# Autodesk Inventor assembly: 42146-10
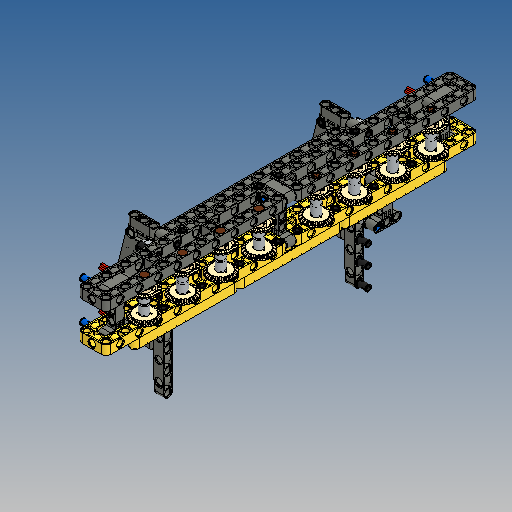
[picture p0: Inventor's stored thumbnail of the model, 512x512]
Saved by Autodesk Inventor 2025 (Build 290162010, 162A)
## iProperties
Created: 2024-11-16
Part Number: 42146-10
Material: Generisch
Document SubType Name: Assembly
Designer: hp.muther
Author: hp.muther
## Documents named in this file (16)
- D:\Inventor\Projekte\Muther\LEGO Technic\LEGO Technik - Raupenkran LR 13000 (42146)\42146-01-10.iam
- D:\Inventor\Projekte\Muther\LEGO Technic\LEGO Pieces\Rahmen, T-Stücke\67491-Yellow.ipt
- D:\Inventor\Projekte\Muther\LEGO Technic\LEGO Pieces\Pin's\6558-Blue.ipt
- D:\Inventor\Projekte\Muther\LEGO Technic\LEGO Pieces\Pin's\11214-Red.ipt
- D:\Inventor\Projekte\Muther\LEGO Technic\LEGO Pieces\Achsen\15462-ReddishBrown.ipt
- D:\Inventor\Projekte\Muther\LEGO Technic\LEGO Pieces\Zahnrad\32198-Tan.ipt
- D:\Inventor\Projekte\Muther\LEGO Technic\LEGO Pieces\Rund\62462-LtBluishGray.ipt
- D:\Inventor\Projekte\Muther\LEGO Technic\LEGO Pieces\Rahmen, T-Stücke\67491-DkBluishGray.ipt
- D:\Inventor\Projekte\Muther\LEGO Technic\LEGO Pieces\Rahmen, T-Stücke\14720-DkBluishGray.ipt
- D:\Inventor\Projekte\Muther\LEGO Technic\LEGO Pieces\Lochbalken\32525-Yellow.ipt
- D:\Inventor\Projekte\Muther\LEGO Technic\LEGO Pieces\Pin's\2780-Black.ipt
- D:\Inventor\Projekte\Muther\LEGO Technic\LEGO Pieces\Pin's\32054-LtBluishGray.ipt
- D:\Inventor\Projekte\Muther\LEGO Technic\LEGO Pieces\Paneelen\18945-DkBluishGray.ipt
- D:\Inventor\Projekte\Muther\LEGO Technic\LEGO Pieces\Pin's\43093-Blue.ipt
- D:\Inventor\Projekte\Muther\LEGO Technic\LEGO Pieces\Lochbalken\43857-LtBluishGray.ipt
- D:\Inventor\Projekte\Muther\LEGO Technic\LEGO Pieces\Lochbalken\771710-DkBluishGray.ipt
## Components (94 placed, 15 different names)
1. 67491-Yellow:1 — Einfügen:1, Einfügen:2, Einfügen:7, Einfügen:8, Einfügen:9, Einfügen:10, Passend:1, Einfügen:23, Einfügen:53, Einfügen:55, Passend:17, Einfügen:56, Passend:18, Einfügen:57, Einfügen:58
2. 6558-Blue:1 — Einfügen:2, Passend:3
3. 11214-Red:1 — Einfügen:1, Passend:2
4. 15462-ReddishBrown:1 — Einfügen:3
5. 32198-Tan:1 — Einfügen:3, Einfügen:10, Einfügen:18
6. 15462-ReddishBrown:2
7. 32198-Tan:2 — Einfügen:9, Einfügen:17
8. 15462-ReddishBrown:3
9. 32198-Tan:3 — Einfügen:8, Einfügen:16
10. 15462-ReddishBrown:4
11. 32198-Tan:4 — Einfügen:7, Einfügen:15
12. 32198-Tan:5 — Einfügen:11
13. 62462-LtBluishGray:1 — Einfügen:11, Einfügen:18
14. 32198-Tan:6
15. 62462-LtBluishGray:2 — Einfügen:17
16. 32198-Tan:7
17. 62462-LtBluishGray:3 — Einfügen:16
18. 32198-Tan:8
19. 62462-LtBluishGray:4 — Einfügen:15
20. 14720-DkBluishGray:1 — Passend:1, Passend:2, Passend:3, Passend:4, Passend:5, Passend:6
21. 67491-DkBluishGray:1 — Passend:4, Passend:7, Passend:19, Einfügen:59, Einfügen:75
22. 6558-Blue:2 — Passend:5
23. 11214-Red:2 — Passend:6
24. 6558-Blue:3 — Einfügen:21, Passend:7, Passend:14
25. 14720-DkBluishGray:2 — Einfügen:21, Einfügen:22, Einfügen:44
26. 6558-Blue:4 — Einfügen:22, Einfügen:23
27. 67491-DkBluishGray:2 — Passend:14, Einfügen:64, Einfügen:82, Einfügen:89
28. 6558-Blue:5
29. 11214-Red:3
30. 15462-ReddishBrown:5
31. 32198-Tan:9
32. 15462-ReddishBrown:6
33. 32198-Tan:10
34. 15462-ReddishBrown:7
35. 32198-Tan:11
36. 15462-ReddishBrown:8
37. 32198-Tan:12
38. 32198-Tan:13
39. 62462-LtBluishGray:5
40. 32198-Tan:14
41. 62462-LtBluishGray:6
42. 32198-Tan:15
43. 62462-LtBluishGray:7
44. 32198-Tan:16
45. 62462-LtBluishGray:8
46. 14720-DkBluishGray:3
47. 67491-Yellow:3 — Einfügen:44, Passend:15, Einfügen:54, Passend:16, Passend:23, Einfügen:90
48. 6558-Blue:6
49. 11214-Red:4
50. 32525-Yellow:1 — Einfügen:49, Einfügen:50, Einfügen:55
51. 32525-Yellow:2 — Einfügen:45, Einfügen:46, Einfügen:47, Einfügen:48, Einfügen:53
52. 2780-Black:1 — Einfügen:50, Passend:17
53. 2780-Black:2 — Einfügen:49
54. 2780-Black:3 — Einfügen:47
55. 2780-Black:4 — Einfügen:46
56. 2780-Black:5 — Einfügen:48
57. 2780-Black:6 — Einfügen:45, Passend:15
58. 2780-Black:7 — Einfügen:59
59. 6558-Blue:7 — Einfügen:58
60. 11214-Red:5 — Einfügen:57
61. 2780-Black:8 — Einfügen:71, Passend:21
62. 2780-Black:9 — Einfügen:78, Passend:22
63. 2780-Black:10 — Einfügen:80
64. 2780-Black:11 — Einfügen:72
65. 2780-Black:12 — Einfügen:69, Passend:20
66. 2780-Black:13 — Einfügen:67
67. 2780-Black:14 — Einfügen:66
68. 2780-Black:15 — Einfügen:68
69. 32054-LtBluishGray:1 — Einfügen:65, Einfügen:74
70. 32525-Yellow:3 — Einfügen:52, Einfügen:54
71. 2780-Black:16 — Einfügen:52
72. 2780-Black:17 — Passend:16
73. 14720-DkBluishGray:4 — Einfügen:56, Passend:18, Einfügen:76
74. 67491-DkBluishGray:3 — Einfügen:60, Einfügen:61, Einfügen:62, Einfügen:63, Einfügen:64
75. 2780-Black:18 — Einfügen:60, Passend:19
76. 2780-Black:19 — Einfügen:63
77. 2780-Black:20 — Einfügen:62
78. 2780-Black:21 — Einfügen:61
79. 771710-DkBluishGray:1 — Einfügen:65, Einfügen:66, Einfügen:67, Einfügen:68, Einfügen:69, Einfügen:70, Einfügen:75, Einfügen:79
80. 32525-Yellow:4 — Einfügen:73, Passend:21
81. 18945-DkBluishGray:1 — Einfügen:70, Passend:20, Einfügen:71, Einfügen:72, Einfügen:73, Passend:22
82. 43093-Blue:1 — Einfügen:74, Einfügen:76
83. 6558-Blue:8 — Einfügen:77
84. 43857-LtBluishGray:1 — Einfügen:77, Einfügen:78, Einfügen:79
85. 771710-DkBluishGray:2 — Einfügen:80, Einfügen:81, Einfügen:82, Einfügen:83, Einfügen:84, Einfügen:85, Einfügen:88
86. 18945-DkBluishGray:2 — Einfügen:85, Passend:24, Passend:25
87. 2780-Black:22 — Einfügen:83
88. 2780-Black:23 — Einfügen:84, Passend:24
89. 6558-Blue:9 — Einfügen:81, Passend:23
90. 2780-Black:24 — Passend:25
91. 6558-Blue:10
92. 43857-LtBluishGray:2 — Einfügen:88
93. 2780-Black:25 — Einfügen:89
94. 2780-Black:26 — Einfügen:90
## Relationships (115: Insert 90, Mate 25)
- Einfügen:1 [Insert]: 67491-Yellow:1 ↔ 11214-Red:1
- Einfügen:2 [Insert]: 67491-Yellow:1 ↔ 6558-Blue:1
- Einfügen:3 [Insert] (7.2 mm): 15462-ReddishBrown:1 ↔ 32198-Tan:1
- [Insert] (7.2 mm): 15462-ReddishBrown:2 ↔ 32198-Tan:2
- [Insert] (7.2 mm): 15462-ReddishBrown:3 ↔ 32198-Tan:3
- [Insert] (7.2 mm): 15462-ReddishBrown:4 ↔ 32198-Tan:4
- Einfügen:7 [Insert]: 67491-Yellow:1 ↔ 32198-Tan:4
- Einfügen:8 [Insert]: 67491-Yellow:1 ↔ 32198-Tan:3
- Einfügen:9 [Insert]: 67491-Yellow:1 ↔ 32198-Tan:2
- Einfügen:10 [Insert]: 67491-Yellow:1 ↔ 32198-Tan:1
- Einfügen:11 [Insert]: 32198-Tan:5 ↔ 62462-LtBluishGray:1
- [Insert]: 32198-Tan:6 ↔ 62462-LtBluishGray:2
- [Insert]: 32198-Tan:7 ↔ 62462-LtBluishGray:3
- [Insert]: 32198-Tan:8 ↔ 62462-LtBluishGray:4
- Einfügen:15 [Insert]: 32198-Tan:4 ↔ 62462-LtBluishGray:4
- Einfügen:16 [Insert]: 32198-Tan:3 ↔ 62462-LtBluishGray:3
- Einfügen:17 [Insert]: 32198-Tan:2 ↔ 62462-LtBluishGray:2
- Einfügen:18 [Insert]: 32198-Tan:1 ↔ 62462-LtBluishGray:1
- Passend:1 [Mate]: 67491-Yellow:1 ↔ 14720-DkBluishGray:1
- Passend:2 [Mate]: 11214-Red:1 ↔ 14720-DkBluishGray:1
- Passend:3 [Mate]: 6558-Blue:1 ↔ 14720-DkBluishGray:1
- [Insert]: 67491-DkBluishGray:1 ↔ 11214-Red:2
- [Insert]: 67491-DkBluishGray:1 ↔ 6558-Blue:2
- Passend:4 [Mate]: 14720-DkBluishGray:1 ↔ 67491-DkBluishGray:1
- Passend:5 [Mate]: 14720-DkBluishGray:1 ↔ 6558-Blue:2
- Passend:6 [Mate]: 14720-DkBluishGray:1 ↔ 11214-Red:2
- Einfügen:21 [Insert]: 6558-Blue:3 ↔ 14720-DkBluishGray:2
- Einfügen:22 [Insert]: 14720-DkBluishGray:2 ↔ 6558-Blue:4
- Einfügen:23 [Insert]: 67491-Yellow:1 ↔ 6558-Blue:4
- Passend:7 [Mate]: 67491-DkBluishGray:1 ↔ 6558-Blue:3
- [Insert]: 67491-DkBluishGray:2 ↔ 11214-Red:3
- [Insert]: 67491-DkBluishGray:2 ↔ 6558-Blue:5
- [Insert] (7.2 mm): 15462-ReddishBrown:5 ↔ 32198-Tan:9
- [Insert] (7.2 mm): 15462-ReddishBrown:6 ↔ 32198-Tan:10
- [Insert] (7.2 mm): 15462-ReddishBrown:7 ↔ 32198-Tan:11
- [Insert] (7.2 mm): 15462-ReddishBrown:8 ↔ 32198-Tan:12
- [Insert]: 67491-DkBluishGray:2 ↔ 32198-Tan:12
- [Insert]: 67491-DkBluishGray:2 ↔ 32198-Tan:11
- [Insert]: 67491-DkBluishGray:2 ↔ 32198-Tan:10
- [Insert]: 67491-DkBluishGray:2 ↔ 32198-Tan:9
- [Insert]: 32198-Tan:13 ↔ 62462-LtBluishGray:5
- [Insert]: 32198-Tan:14 ↔ 62462-LtBluishGray:6
- [Insert]: 32198-Tan:15 ↔ 62462-LtBluishGray:7
- [Insert]: 32198-Tan:16 ↔ 62462-LtBluishGray:8
- [Insert]: 32198-Tan:12 ↔ 62462-LtBluishGray:8
- [Insert]: 32198-Tan:11 ↔ 62462-LtBluishGray:7
- [Insert]: 32198-Tan:10 ↔ 62462-LtBluishGray:6
- [Insert]: 32198-Tan:9 ↔ 62462-LtBluishGray:5
- [Mate]: 67491-DkBluishGray:2 ↔ 14720-DkBluishGray:3
- [Mate]: 11214-Red:3 ↔ 14720-DkBluishGray:3
- [Mate]: 6558-Blue:5 ↔ 14720-DkBluishGray:3
- [Insert]: 67491-Yellow:3 ↔ 11214-Red:4
- [Insert]: 67491-Yellow:3 ↔ 6558-Blue:6
- [Mate]: 14720-DkBluishGray:3 ↔ 67491-Yellow:3
- [Mate]: 14720-DkBluishGray:3 ↔ 6558-Blue:6
- [Mate]: 14720-DkBluishGray:3 ↔ 11214-Red:4
- Einfügen:44 [Insert]: 14720-DkBluishGray:2 ↔ 67491-Yellow:3
- Passend:14 [Mate]: 6558-Blue:3 ↔ 67491-DkBluishGray:2
- Einfügen:45 [Insert]: 32525-Yellow:2 ↔ 2780-Black:6
- Einfügen:46 [Insert]: 32525-Yellow:2 ↔ 2780-Black:4
- Einfügen:47 [Insert]: 32525-Yellow:2 ↔ 2780-Black:3
- Einfügen:48 [Insert]: 32525-Yellow:2 ↔ 2780-Black:5
- Einfügen:49 [Insert]: 32525-Yellow:1 ↔ 2780-Black:2
- Einfügen:50 [Insert]: 32525-Yellow:1 ↔ 2780-Black:1
- [Insert]: 32525-Yellow:3 ↔ 2780-Black:17
- Einfügen:52 [Insert]: 32525-Yellow:3 ↔ 2780-Black:16
- Einfügen:53 [Insert]: 67491-Yellow:1 ↔ 32525-Yellow:2
- Passend:15 [Mate]: 67491-Yellow:3 ↔ 2780-Black:6
- Einfügen:54 [Insert]: 67491-Yellow:3 ↔ 32525-Yellow:3
- Passend:16 [Mate]: 67491-Yellow:3 ↔ 2780-Black:17
- Einfügen:55 [Insert]: 67491-Yellow:1 ↔ 32525-Yellow:1
- Passend:17 [Mate]: 67491-Yellow:1 ↔ 2780-Black:1
- Einfügen:56 [Insert]: 67491-Yellow:1 ↔ 14720-DkBluishGray:4
- Passend:18 [Mate]: 67491-Yellow:1 ↔ 14720-DkBluishGray:4
- Einfügen:57 [Insert]: 67491-Yellow:1 ↔ 11214-Red:5
- Einfügen:58 [Insert]: 67491-Yellow:1 ↔ 6558-Blue:7
- Einfügen:59 [Insert]: 67491-DkBluishGray:1 ↔ 2780-Black:7
- Einfügen:60 [Insert]: 67491-DkBluishGray:3 ↔ 2780-Black:18
- Einfügen:61 [Insert]: 67491-DkBluishGray:3 ↔ 2780-Black:21
- Einfügen:62 [Insert]: 67491-DkBluishGray:3 ↔ 2780-Black:20
- Einfügen:63 [Insert]: 67491-DkBluishGray:3 ↔ 2780-Black:19
- Einfügen:64 [Insert]: 67491-DkBluishGray:2 ↔ 67491-DkBluishGray:3
- Passend:19 [Mate]: 67491-DkBluishGray:1 ↔ 2780-Black:18
- Einfügen:65 [Insert]: 32054-LtBluishGray:1 ↔ 771710-DkBluishGray:1
- Einfügen:66 [Insert]: 2780-Black:14 ↔ 771710-DkBluishGray:1
- Einfügen:67 [Insert]: 2780-Black:13 ↔ 771710-DkBluishGray:1
- Einfügen:68 [Insert]: 2780-Black:15 ↔ 771710-DkBluishGray:1
- Einfügen:69 [Insert]: 2780-Black:12 ↔ 771710-DkBluishGray:1
- Einfügen:70 [Insert]: 771710-DkBluishGray:1 ↔ 18945-DkBluishGray:1
- Passend:20 [Mate]: 2780-Black:12 ↔ 18945-DkBluishGray:1
- Einfügen:71 [Insert]: 2780-Black:8 ↔ 18945-DkBluishGray:1
- Einfügen:72 [Insert]: 2780-Black:11 ↔ 18945-DkBluishGray:1
- Einfügen:73 [Insert]: 32525-Yellow:4 ↔ 18945-DkBluishGray:1
- Passend:21 [Mate]: 2780-Black:8 ↔ 32525-Yellow:4
- Einfügen:74 [Insert]: 32054-LtBluishGray:1 ↔ 43093-Blue:1
- Einfügen:75 [Insert]: 67491-DkBluishGray:1 ↔ 771710-DkBluishGray:1
- Einfügen:76 [Insert]: 14720-DkBluishGray:4 ↔ 43093-Blue:1
- Einfügen:77 [Insert]: 6558-Blue:8 ↔ 43857-LtBluishGray:1
- Einfügen:78 [Insert]: 2780-Black:9 ↔ 43857-LtBluishGray:1
- Einfügen:79 [Insert]: 771710-DkBluishGray:1 ↔ 43857-LtBluishGray:1
- Passend:22 [Mate]: 2780-Black:9 ↔ 18945-DkBluishGray:1
- Einfügen:80 [Insert]: 2780-Black:10 ↔ 771710-DkBluishGray:2
- Einfügen:81 [Insert]: 771710-DkBluishGray:2 ↔ 6558-Blue:9
- Einfügen:82 [Insert]: 67491-DkBluishGray:2 ↔ 771710-DkBluishGray:2
- Passend:23 [Mate]: 67491-Yellow:3 ↔ 6558-Blue:9
- Einfügen:83 [Insert]: 771710-DkBluishGray:2 ↔ 2780-Black:22
- Einfügen:84 [Insert]: 771710-DkBluishGray:2 ↔ 2780-Black:23
- Einfügen:85 [Insert]: 771710-DkBluishGray:2 ↔ 18945-DkBluishGray:2
- Passend:24 [Mate]: 18945-DkBluishGray:2 ↔ 2780-Black:23
- [Insert]: 6558-Blue:10 ↔ 43857-LtBluishGray:2
- [Insert]: 2780-Black:24 ↔ 43857-LtBluishGray:2
- Einfügen:88 [Insert]: 771710-DkBluishGray:2 ↔ 43857-LtBluishGray:2
- Passend:25 [Mate]: 18945-DkBluishGray:2 ↔ 2780-Black:24
- Einfügen:89 [Insert]: 67491-DkBluishGray:2 ↔ 2780-Black:25
- Einfügen:90 [Insert]: 67491-Yellow:3 ↔ 2780-Black:26
## Named parameters: d3_d2 = 7.2 mm, d4_d2 = 7.2 mm, d5_d2 = 7.2 mm, d11_d10 = 0 mm, d12_d10 = 0 mm, d13_d10 = 0 mm, d21_d0 = 0 mm, d22_d1 = 0 mm, d26_d20 = 0 mm, d27_d24 = 0 mm, d30_d2 = 7.2 mm, d31_d3_d2 = 7.2 mm, d32_d4_d2 = 7.2 mm, d33_d5_d2 = 7.2 mm, d34_d6 = 0 mm, d35_d7 = 0 mm, d36_d8 = 0 mm, d37_d9 = 0 mm, d38_d10 = 0 mm, d39_d11_d10 = 0 mm, d40_d12_d10 = 0 mm, d41_d13_d10 = 0 mm, d42_d14 = 0 mm, d43_d15 = 0 mm, d44_d16 = 0 mm, d45_d17 = 0 mm, d46_d18 = 0 mm, d47_d19 = 0 mm, d48_d20 = 0 mm, d49_d21_d0 = 0 mm, d50_d22_d1 = 0 mm, d51_d23 = 0 mm, d52_d24 = 0 mm, d53_d25 = 0 mm, d54_d0 = 0 mm, d55_d1 = 0 mm, d64_d62 = 0 mm, d65_d63 = 0 mm, d110_d97 = 0 mm, d111_d98 = 0 mm
